# Autodesk Inventor assembly: Product_PipeShoe
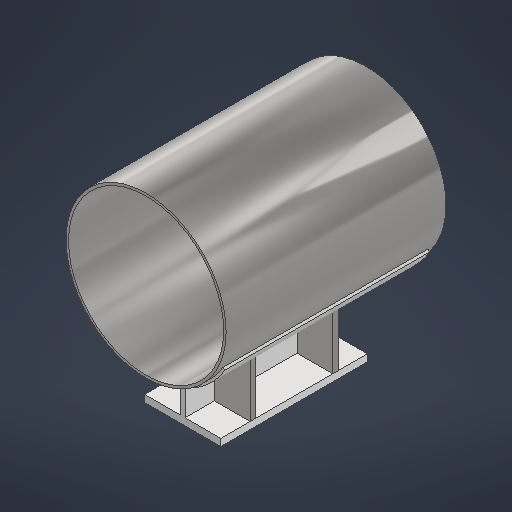
[picture p0: Inventor's stored thumbnail of the model, 512x512]
Saved by Autodesk Inventor 2025 (Build 290162000, 162)
## iProperties
Created: 2024-06-07
Part Number: Product_PipeShoe
Document SubType Name: Assembly
Designer: a0976
Author: a0976
## Documents named in this file (6)
- C:\Users\a0976\Desktop\testing\Product_PipeShoe.iam
- C:\Users\a0976\Desktop\testing\A.ipt
- C:\Users\a0976\Desktop\testing\B.ipt
- C:\Users\a0976\Desktop\testing\C.ipt
- C:\Users\a0976\Desktop\testing\D.ipt
- C:\Users\a0976\Desktop\testing\D_MIR.ipt
## Components (7 placed, 5 different names)
1. A:1 — 齊平:6, 齊平:7, 貼合:2, 齊平:8, 貼合:3, 貼合:4, 齊平:9, 齊平:10, 貼合:5
2. B:1 — 貼合:1, 齊平:4, 齊平:5
3. C:1 — 齊平:1, 齊平:2, 齊平:3, 貼合:1, 貼合:2
4. D:1 — 齊平:8, 貼合:3, 貼合:4
5. D:2 — 齊平:9, 齊平:10, 貼合:5
6. D_MIR:1
7. D_MIR:2
## Relationships (15: Flush 10, Mate 5)
- 齊平:1 [Flush]: C:1
- 齊平:2 [Flush]: C:1
- 齊平:3 [Flush]: C:1
- 貼合:1 [Mate]: B:1 ↔ C:1
- 齊平:4 [Flush]: B:1
- 齊平:5 [Flush]: B:1
- 齊平:6 [Flush]: A:1
- 齊平:7 [Flush]: A:1
- 貼合:2 [Mate]: A:1 ↔ C:1
- 齊平:8 [Flush] (50 mm): A:1 ↔ D:1
- 貼合:3 [Mate]: A:1 ↔ D:1
- 貼合:4 [Mate]: A:1 ↔ D:1
- 齊平:9 [Flush] (50 mm): A:1 ↔ D:2
- 齊平:10 [Flush]: A:1 ↔ D:2
- 貼合:5 [Mate]: A:1 ↔ D:2
## Named parameters: lineSize = 10, Scthick = 10, Section_buttom_A = 130 mm, Extra_Plate_B = 9 mm, another_Section_buttom = 200 mm, Extra_Lops = 250 mm, The_Gap_for_section = 50 mm
